# Autodesk Inventor assembly: Fly Wheel SubAssembly
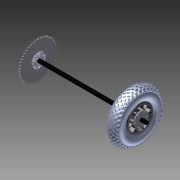
[picture p0: Inventor's stored thumbnail of the model, 180x180]
Saved by Autodesk Inventor 2014 SP1 (Build 180222100, 222)
## iProperties
Created: 2014-01-20
Part Number: Fly Wheel SubAssembly
Document SubType Name: Assembly
Designer: Paul
Author: Paul
## Documents named in this file (6)
- C:\FRC_CAD\4859cad\Robot\Actual Robot\Fly Wheel\Fly Wheel SubAssembly.iam
- C:\FRC_CAD\4859cad\Robot\Actual Robot\Fly Wheel\Imported Components\PneumaticWheel_am-0970\PneumaticWheel_am-0970.iam
- C:\FRC_CAD\4859cad\Robot\Drivetrain\Imported Components\Hex Versa Hub\Hex Versa Hub.ipt
- C:\FRC_CAD\4859cad\Robot\Actual Robot\Fly Wheel\Imported Components\Imported Components\500_hex_hub\500_hex_hub.ipt
- C:\FRC_CAD\4859cad\Robot\Actual Robot\Fly Wheel\Half Inch Hex Stock.ipt
- C:\FRC_CAD\4859cad\Robot\Actual Robot\Fly Wheel\Imported Components\#35 Sprocket 48t\#35 Sprocket 48t.ipt
## Components (6 placed, 5 different names)
1. PneumaticWheel_am-0970:1 [sub-assembly] — Mate:1, Mate:2, Mate:3, Mate:4, Mate:5, Mate:6
2. 500_hex_hub:1 — Mate:1, Mate:2, Mate:3, Flush:1
3. 500_hex_hub:2 — Mate:4, Mate:5, Mate:6, Mate:7, Mate:8
4. Half Inch Hex Stock:1 — Mate:7, Mate:8, Flush:1, Mate:11, Mate:12, Flush:2
5. #35 Sprocket 48t:1 — Mate:13, Mate:14
6. Hex Versa Hub:1 — Mate:11, Mate:12, Flush:2, Mate:13, Mate:14
## Relationships (14: Mate 12, Flush 2)
- Mate:1: PneumaticWheel_am-0970:1 ↔ 500_hex_hub:1
- Mate:2: PneumaticWheel_am-0970:1 ↔ 500_hex_hub:1
- Mate:3: PneumaticWheel_am-0970:1 ↔ 500_hex_hub:1
- Mate:4: PneumaticWheel_am-0970:1 ↔ 500_hex_hub:2
- Mate:5: PneumaticWheel_am-0970:1 ↔ 500_hex_hub:2
- Mate:6: PneumaticWheel_am-0970:1 ↔ 500_hex_hub:2
- Mate:7: 500_hex_hub:2 ↔ Half Inch Hex Stock:1
- Mate:8: 500_hex_hub:2 ↔ Half Inch Hex Stock:1
- Flush:1 (23.495 mm): 500_hex_hub:1 ↔ Half Inch Hex Stock:1
- Mate:11: Half Inch Hex Stock:1 ↔ Hex Versa Hub:1
- Mate:12: Half Inch Hex Stock:1 ↔ Hex Versa Hub:1
- Flush:2 (12.7 mm): Half Inch Hex Stock:1 ↔ Hex Versa Hub:1
- Mate:13: #35 Sprocket 48t:1 ↔ Hex Versa Hub:1
- Mate:14: #35 Sprocket 48t:1 ↔ Hex Versa Hub:1
